# Autodesk Inventor assembly: Mais uma montagem
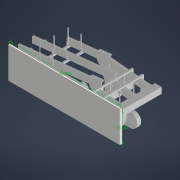
[picture p0: Inventor's stored thumbnail of the model, 180x180]
Saved by Autodesk Inventor 2022 (Build 260153000, 153)
## iProperties
Created: 2023-05-12
Part Number: Mais uma montagem
Document SubType Name: Assembly
Designer: jpjoa
Author: jpjoa
## Documents named in this file (16)
- G:\My Drive\Faculdade\Trabalhos\Desenho e Print 3D\Marbles project\Mais uma montagem.iam
- G:\My Drive\Faculdade\Trabalhos\Desenho e Print 3D\Marbles project\Base.ipt
- G:\My Drive\Faculdade\Trabalhos\Desenho e Print 3D\Marbles project\Box de reinício.ipt
- G:\My Drive\Faculdade\Trabalhos\Desenho e Print 3D\Marbles project\Conector superior para giro.ipt
- G:\My Drive\Faculdade\Trabalhos\Desenho e Print 3D\Marbles project\Libera todas.ipt
- G:\My Drive\Faculdade\Trabalhos\Desenho e Print 3D\Marbles project\Parafuso.ipt
- G:\My Drive\Faculdade\Trabalhos\Desenho e Print 3D\Marbles project\Pega uma e libera superior.ipt
- G:\My Drive\Faculdade\Trabalhos\Desenho e Print 3D\Marbles project\Pega uma e libera.ipt
- G:\My Drive\Faculdade\Trabalhos\Desenho e Print 3D\Marbles project\Receptor pequeno.ipt
- G:\My Drive\Faculdade\Trabalhos\Desenho e Print 3D\Marbles project\Receptor.ipt
- G:\My Drive\Faculdade\Trabalhos\Desenho e Print 3D\Marbles project\Sustentação Trilhos fixos.ipt
- G:\My Drive\Faculdade\Trabalhos\Desenho e Print 3D\Marbles project\Sustentação Trilhos.ipt
- G:\My Drive\Faculdade\Trabalhos\Desenho e Print 3D\Marbles project\Trilho 5 minutos.ipt
- G:\My Drive\Faculdade\Trabalhos\Desenho e Print 3D\Marbles project\Trilho 60 minutos  - 12 horas.ipt
- G:\My Drive\Faculdade\Trabalhos\Desenho e Print 3D\Marbles project\Troca de sentido.ipt
- G:\My Drive\Faculdade\Trabalhos\Desenho e Print 3D\Marbles project\Agrupar bolinhas novamente.ipt
## Components (30 placed, 15 different names)
1. Base:1 — Alinhado:2, Coincidente:1, Coincidente:3, Alinhado:14, Coincidente:12, Coincidente:13, Coincidente:14, Coincidente:16
2. Box de reinício:1 — Alinhado:2, Coincidente:1, Coincidente:4, Alinhado:15, Inserir:7, Inserir:8, Inserir:9, Alinhado:21, Coincidente:19, Inserir:26
3. Conector superior para giro:1 — Inserir:4
4. Libera todas:1 — Alinhado:11, Alinhado:13, Inserir:7
5. Pega uma e libera superior:1 — Alinhado:13, Alinhado:15, Inserir:8, Coincidente:8, Alinhado:18, Coincidente:9
6. Pega uma e libera:1 — Alinhado:11, Alinhado:17, Inserir:9, Coincidente:10, Coincidente:11, Coincidente:20
7. Receptor pequeno:1 — Alinhado:17, Alinhado:19, Coincidente:10, Coincidente:11, Coincidente:20
8. Sustentação Trilhos fixos:1 — Coincidente:3, Coincidente:4, Alinhado:14, Alinhado:20, Rígida:1, Inserir:10, Inserir:11, Inserir:12, Inserir:13, Inserir:14, Coincidente:15, Alinhado:22
9. Sustentação Trilhos:1 — Coincidente:16, Coincidente:17, Inserir:18, Inserir:19, Inserir:20, Inserir:21, Inserir:22, Inserir:23, Coincidente:18, Coincidente:19
10. Trilho 5 minutos:1 — Inserir:5, Alinhado:6, Coincidente:17, Tangente:1, Tangente:4
11. Troca de sentido:1 — Inserir:4
12. Receptor:3 — Inserir:5, Alinhado:6, Alinhado:24
13. Receptor pequeno:2 — Coincidente:8, Alinhado:18, Coincidente:9, Alinhado:19
14. Parafuso:2 — Inserir:10
15. Parafuso:3 — Inserir:11
16. Parafuso:4 — Inserir:12
17. Parafuso:5 — Inserir:13
18. Parafuso:6 — Alinhado:20, Rígida:1
19. Parafuso:7 — Inserir:14
20. Parafuso:8 — Inserir:22, Tangente:5
21. Parafuso:9 — Inserir:21, Tangente:3
22. Parafuso:10 — Inserir:18, Tangente:1
23. Parafuso:11 — Inserir:23, Tangente:6
24. Parafuso:12 — Inserir:20, Tangente:2
25. Parafuso:13 — Inserir:19, Tangente:4
26. Trilho 60 minutos  - 12 horas:1 — Inserir:24, Tangente:2, Tangente:5
27. Trilho 60 minutos  - 12 horas:2 — Inserir:25, Tangente:3, Tangente:6
28. Receptor:4 — Inserir:24, Alinhado:23, Alinhado:24
29. Receptor:5 — Inserir:25, Alinhado:23
30. Agrupar bolinhas novamente:1 — Inserir:26
## Relationships (56: Insert 19, Mate 16, Flush 14, Tangent 6, WeldJoint 1)
- Alinhado:2 [Flush]: Base:1 ↔ Box de reinício:1
- Coincidente:1 [Mate]: Base:1 ↔ Box de reinício:1
- Inserir:4: Conector superior para giro:1 ↔ Troca de sentido:1
- Inserir:5: Trilho 5 minutos:1 ↔ Receptor:3
- Alinhado:6 [Flush]: Trilho 5 minutos:1 ↔ Receptor:3
- Coincidente:3 [Mate]: Base:1 ↔ Sustentação Trilhos fixos:1
- Alinhado:11 [Flush]: Libera todas:1 ↔ Pega uma e libera:1
- Alinhado:13 [Flush]: Libera todas:1 ↔ Pega uma e libera superior:1
- Coincidente:4 [Mate]: Box de reinício:1 ↔ Sustentação Trilhos fixos:1
- Alinhado:14 [Flush]: Base:1 ↔ Sustentação Trilhos fixos:1
- Alinhado:15 [Flush]: Box de reinício:1 ↔ Pega uma e libera superior:1
- Alinhado:17 [Flush]: Pega uma e libera:1 ↔ Receptor pequeno:1
- Inserir:7: Box de reinício:1 ↔ Libera todas:1
- Inserir:8: Box de reinício:1 ↔ Pega uma e libera superior:1
- Inserir:9: Box de reinício:1 ↔ Pega uma e libera:1
- Coincidente:8 [Mate]: Pega uma e libera superior:1 ↔ Receptor pequeno:2
- Alinhado:18 [Flush]: Pega uma e libera superior:1 ↔ Receptor pequeno:2
- Coincidente:9 [Mate]: Pega uma e libera superior:1 ↔ Receptor pequeno:2
- Alinhado:19 [Flush]: Receptor pequeno:1 ↔ Receptor pequeno:2
- Coincidente:10 [Mate]: Pega uma e libera:1 ↔ Receptor pequeno:1
- Coincidente:11 [Mate]: Pega uma e libera:1 ↔ Receptor pequeno:1
- Coincidente:12 [Mate]: Base:1
- Coincidente:13 [Mate]: Base:1
- Coincidente:14 [Mate]: Base:1
- Alinhado:20 [Flush]: Sustentação Trilhos fixos:1 ↔ Parafuso:6
- Rígida:1 [WeldJoint]: Sustentação Trilhos fixos:1 ↔ Parafuso:6
- Inserir:10: Sustentação Trilhos fixos:1 ↔ Parafuso:2
- Inserir:11: Sustentação Trilhos fixos:1 ↔ Parafuso:3
- Inserir:12: Sustentação Trilhos fixos:1 ↔ Parafuso:4
- Inserir:13: Sustentação Trilhos fixos:1 ↔ Parafuso:5
- Inserir:14: Sustentação Trilhos fixos:1 ↔ Parafuso:7
- Alinhado:21 [Flush] (73.935 mm): Box de reinício:1
- Coincidente:15 [Mate]: Sustentação Trilhos fixos:1
- Coincidente:16 [Mate]: Base:1 ↔ Sustentação Trilhos:1
- Coincidente:17 [Mate]: Sustentação Trilhos:1 ↔ Trilho 5 minutos:1
- Inserir:18: Sustentação Trilhos:1 ↔ Parafuso:10
- Inserir:19: Sustentação Trilhos:1 ↔ Parafuso:13
- Inserir:20: Sustentação Trilhos:1 ↔ Parafuso:12
- Inserir:21: Sustentação Trilhos:1 ↔ Parafuso:9
- Inserir:22: Sustentação Trilhos:1 ↔ Parafuso:8
- Inserir:23: Sustentação Trilhos:1 ↔ Parafuso:11
- Tangente:1: Trilho 5 minutos:1 ↔ Parafuso:10
- Alinhado:22 [Flush] (156.718 mm): Sustentação Trilhos fixos:1
- Coincidente:18 [Mate]: Sustentação Trilhos:1
- Inserir:24: Trilho 60 minutos  - 12 horas:1 ↔ Receptor:4
- Inserir:25: Trilho 60 minutos  - 12 horas:2 ↔ Receptor:5
- Alinhado:23 [Flush]: Receptor:4 ↔ Receptor:5
- Alinhado:24 [Flush]: Receptor:3 ↔ Receptor:4
- Tangente:2: Parafuso:12 ↔ Trilho 60 minutos  - 12 horas:1
- Tangente:3: Parafuso:9 ↔ Trilho 60 minutos  - 12 horas:2
- Tangente:4: Trilho 5 minutos:1 ↔ Parafuso:13
- Coincidente:19 [Mate]: Box de reinício:1 ↔ Sustentação Trilhos:1
- Tangente:5: Parafuso:8 ↔ Trilho 60 minutos  - 12 horas:1
- Tangente:6: Parafuso:11 ↔ Trilho 60 minutos  - 12 horas:2
- Coincidente:20 [Mate]: Pega uma e libera:1 ↔ Receptor pequeno:1
- Inserir:26: Box de reinício:1 ↔ Agrupar bolinhas novamente:1
